# Autodesk Inventor assembly: workshop
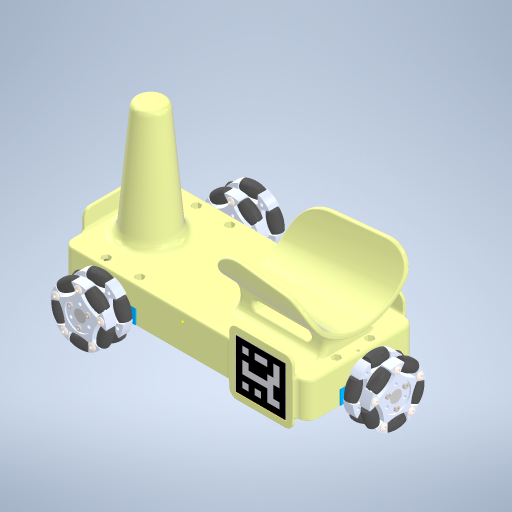
[picture p0: Inventor's stored thumbnail of the model, 512x512]
Saved by Autodesk Inventor 2024 (Build 280153000, 153)
## iProperties
Created: 2024-02-01
Part Number: workshop
Document SubType Name: Assembly
Designer: Pintu
Author: Pintu
## Documents named in this file (11)
- D:\CMC\my_inventor\ArmBo_v2\workshop.iam
- D:\CMC\my_inventor\ArmBo_v2\hand_rest_v4.ipt
- D:\CMC\my_inventor\ArmBo_v2\new_shaft.ipt
- D:\CMC\my_inventor\ArmBo_v2\workshop\Design Accelerator\Bearing1.iam
- D:\CMC\my_inventor\ArmBo_v2\workshop\Design Accelerator\Bearing2.iam
- D:\CMC\my_inventor\ArmBo_v2\workshop\Design Accelerator\Bearing3.iam
- D:\CMC\my_inventor\ArmBo_v2\bearing_holder_v3.ipt
- C:\Users\Pintu\Documents\Inventor\Content Center Files\R2024\en-US\ISO 4762(2)\ISO 4762 - M4 x 30ISO.ipt
- C:\Users\Pintu\Documents\Inventor\Content Center Files\R2024\en-US\ISO 8738(2)\ISO 8738 - 4(2).ipt
- C:\Users\Pintu\Documents\Inventor\Content Center Files\R2024\en-US\ISO 4035(2)\ISO 4035 - M4 - ISO.ipt
- D:\CMC\my_inventor\ArmBo_v2\support\WheelAsm\WheelAsm.iam
## Components (16 placed, 8 different names)
1. hand_rest_v4:1 — Mate:1, Mate:2, Mate:3, Mate:5, Mate:7, Mate:9, Mate:12, Mate:13, Mate:14, Mate:15, Mate:16, Mate:17, Mate:18, Mate:20, Mate:21, Mate:25, Mate:26, Mate:27, Mate:28
2. new_shaft:1 — Mate:2, Mate:4, Mate:6, Mate:13, Mate:23, Flush:2
3. new_shaft:2 — Mate:1, Mate:14, Mate:22, Rotation:1, Flush:1
4. new_shaft:3 — Mate:3, Mate:8, Mate:12, Mate:24, Flush:3
5. Bearing:1 [sub-assembly] — Mate:4, Mate:5
6. Bearing:2 [sub-assembly] — Mate:6, Mate:7
7. Bearing:3 [sub-assembly] — Mate:8, Mate:9
8. bearing_holder_v3:1 — Mate:15, Mate:16, Mate:17, Mate:19
9. bearing_holder_v3:3 — Mate:25, Mate:26
10. ISO 4762 M4 x 30:1 — Mate:18, Mate:19
11. ISO 8738 4:1 — Mate:20, Mate:21, Insert:1
12. ISO 4035 M4:1 — Insert:1
13. WheelAsm:1 [sub-assembly] — Mate:22, Rotation:1, Flush:1
14. WheelAsm:2 [sub-assembly] — Mate:23, Flush:2
15. WheelAsm:3 [sub-assembly] — Mate:24, Flush:3
16. bearing_holder_v3:4 — Mate:27, Mate:28
## Relationships (31: Mate 26, Flush 3, Insert 1, RelateRotation 1)
- Mate:1: hand_rest_v4:1 ↔ new_shaft:2
- Mate:2: hand_rest_v4:1 ↔ new_shaft:1
- Mate:3: hand_rest_v4:1 ↔ new_shaft:3
- Mate:4: new_shaft:1 ↔ Bearing:1
- Mate:5: hand_rest_v4:1 ↔ Bearing:1
- Mate:6: new_shaft:1 ↔ Bearing:2
- Mate:7: hand_rest_v4:1 ↔ Bearing:2
- Mate:8: new_shaft:3 ↔ Bearing:3
- Mate:9: hand_rest_v4:1 ↔ Bearing:3
- Mate:12: hand_rest_v4:1 ↔ new_shaft:3
- Mate:13: hand_rest_v4:1 ↔ new_shaft:1
- Mate:14: hand_rest_v4:1 ↔ new_shaft:2
- Mate:15: hand_rest_v4:1 ↔ bearing_holder_v3:1
- Mate:16 (1 mm): hand_rest_v4:1 ↔ bearing_holder_v3:1
- Mate:17: hand_rest_v4:1 ↔ bearing_holder_v3:1
- Mate:18: hand_rest_v4:1 ↔ ISO 4762 M4 x 30:1
- Mate:19: bearing_holder_v3:1 ↔ ISO 4762 M4 x 30:1
- Mate:20: hand_rest_v4:1 ↔ ISO 8738 4:1
- Mate:21: hand_rest_v4:1 ↔ ISO 8738 4:1
- Insert:1: ISO 8738 4:1 ↔ ISO 4035 M4:1
- Mate:22: new_shaft:2 ↔ WheelAsm:1
- Mate:23: new_shaft:1 ↔ WheelAsm:2
- Mate:24: new_shaft:3 ↔ WheelAsm:3
- Rotation:1 [RelateRotation] (1 ul): new_shaft:2 ↔ WheelAsm:1
- Flush:1: new_shaft:2 ↔ WheelAsm:1
- Flush:2: new_shaft:1 ↔ WheelAsm:2
- Flush:3: new_shaft:3 ↔ WheelAsm:3
- Mate:25: hand_rest_v4:1 ↔ bearing_holder_v3:3
- Mate:26: hand_rest_v4:1 ↔ bearing_holder_v3:3
- Mate:27: hand_rest_v4:1 ↔ bearing_holder_v3:4
- Mate:28: hand_rest_v4:1 ↔ bearing_holder_v3:4
